# Autodesk Inventor assembly: moving fighting bot
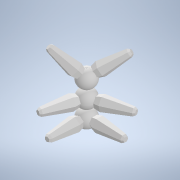
[picture p0: Inventor's stored thumbnail of the model, 180x180]
Saved by Autodesk Inventor 2022 (Build 260153000, 153)
## iProperties
Created: 2022-03-14
Part Number: moving fighting bot
Document SubType Name: Assembly
Designer: mogje
Author: mogje
## Documents named in this file (8)
- D:\Program Files (x86)\Autodesk Inventor\Projects\Microbots\moving fighting bot.iam
- D:\Program Files (x86)\Autodesk Inventor\Projects\Microbots\arm rings.ipt
- D:\Program Files (x86)\Autodesk Inventor\Projects\Microbots\ball tops.ipt
- D:\Program Files (x86)\Autodesk Inventor\Projects\Microbots\bottom ball bottom.ipt
- D:\Program Files (x86)\Autodesk Inventor\Projects\Microbots\mid ball bottom.ipt
- D:\Program Files (x86)\Autodesk Inventor\Projects\Microbots\head mount ring.ipt
- D:\Program Files (x86)\Autodesk Inventor\Projects\Microbots\bulb turning point.ipt
- D:\Program Files (x86)\Autodesk Inventor\Projects\Microbots\arms.ipt
## Components (17 placed, 7 different names)
1. arm rings:1 — Mate:11, Mate:14, Mate:23, Mate:28
2. arm rings:2 — Mate:9, Mate:10, Mate:26, Mate:31
3. arm rings:3 — Mate:1, Mate:2, Mate:21, Mate:22
4. arm rings:4 — Mate:3, Mate:6, Mate:25, Mate:32
5. ball tops:1 — Mate:12, Mate:13, Mate:14, Mate:19, Mate:20
6. ball tops:2 — Mate:4, Mate:5, Mate:6, Mate:7, Mate:8
7. bottom ball bottom:1 — Mate:1, Mate:2, Mate:3, Mate:4, Mate:5
8. mid ball bottom:1 — Mate:7, Mate:8, Mate:9, Mate:10, Mate:11, Mate:12, Mate:13
9. head mount ring:1 — Mate:15, Mate:16, Mate:17, Mate:18, Mate:19, Mate:20
10. head bulb:1 — Mate:15, Mate:16, Mate:24, Mate:29
11. head bulb:2 — Mate:17, Mate:18, Mate:27, Mate:30
12. arms:1 — Mate:26, Mate:31
13. arms:2 — Mate:25, Mate:32
14. arms:3 — Mate:27, Mate:30
15. arms:4 — Mate:24, Mate:29
16. arms:5 — Mate:23, Mate:28
17. arms:6 — Mate:21, Mate:22
## Relationships (32: Mate 32)
- Mate:1: arm rings:3 ↔ bottom ball bottom:1
- Mate:2: arm rings:3 ↔ bottom ball bottom:1
- Mate:3: arm rings:4 ↔ bottom ball bottom:1
- Mate:4: ball tops:2 ↔ bottom ball bottom:1
- Mate:5: ball tops:2 ↔ bottom ball bottom:1
- Mate:6: arm rings:4 ↔ ball tops:2
- Mate:7: ball tops:2 ↔ mid ball bottom:1
- Mate:8: ball tops:2 ↔ mid ball bottom:1
- Mate:9: arm rings:2 ↔ mid ball bottom:1
- Mate:10: arm rings:2 ↔ mid ball bottom:1
- Mate:11: arm rings:1 ↔ mid ball bottom:1
- Mate:12: ball tops:1 ↔ mid ball bottom:1
- Mate:13: ball tops:1 ↔ mid ball bottom:1
- Mate:14: arm rings:1 ↔ ball tops:1
- Mate:15: head mount ring:1 ↔ head bulb:1
- Mate:16: head mount ring:1 ↔ head bulb:1
- Mate:17: head mount ring:1 ↔ head bulb:2
- Mate:18: head mount ring:1 ↔ head bulb:2
- Mate:19: ball tops:1 ↔ head mount ring:1
- Mate:20: ball tops:1 ↔ head mount ring:1
- Mate:21: arm rings:3 ↔ arms:6
- Mate:22: arm rings:3 ↔ arms:6
- Mate:23: arm rings:1 ↔ arms:5
- Mate:24: head bulb:1 ↔ arms:4
- Mate:25: arm rings:4 ↔ arms:2
- Mate:26: arm rings:2 ↔ arms:1
- Mate:27: head bulb:2 ↔ arms:3
- Mate:28: arm rings:1 ↔ arms:5
- Mate:29: head bulb:1 ↔ arms:4
- Mate:30: head bulb:2 ↔ arms:3
- Mate:31: arm rings:2 ↔ arms:1
- Mate:32: arm rings:4 ↔ arms:2
